# Autodesk Inventor assembly: Traction_Section_MIR2
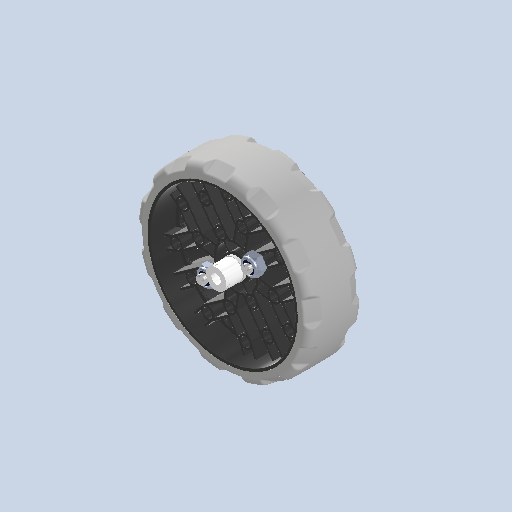
[picture p0: Inventor's stored thumbnail of the model, 512x512]
Saved by Autodesk Inventor 2025.2 (Build 292293000, 293)
## iProperties
Created: 2024-12-08
Part Number: Traction_Section_MIR2
Document SubType Name: Assembly
Designer: joshi
Author: Aditya Koduri
## Documents named in this file (11)
- C:\Users\joshi\Desktop\3388K CAD\Traction_Section_MIR2.iam
- C:\Users\joshi\Desktop\3388K CAD\VEX Main\Motion\Gears\HS Gear\HS 48T Gear, No Insert_MIR2.iam
- C:\Users\joshi\Desktop\3388K CAD\VEX Main\Structure\Hardware\Nut Thin Nylock_MIR2.ipt
- C:\Users\joshi\Desktop\3388K CAD\VEX Main\Motion\Insert Circle_MIR2.ipt
- C:\Users\joshi\Desktop\3388K CAD\VEX Main\Motion\Spacers\Washer Teflon\TWasher .375 OD x .03125.ipt
- C:\Users\joshi\Desktop\3388K CAD\VEX Main\Motion\Spacers\Washer Teflon.ipt
- C:\Users\joshi\Desktop\3388K CAD\VEX Main\Motion\Spacers\Spacer Nylon .313 OD\NSpacer .313 OD x .250.ipt
- C:\Users\joshi\Desktop\3388K CAD\VEX Main\Motion\Spacers\Spacer Nylon .313 OD.ipt
- C:\Users\joshi\Desktop\3388K CAD\VEX Main\Motion\Wheels\Traction Wheel\3.25 Traction AS, No Insert_MIR2.iam
- C:\Users\joshi\Desktop\3388K CAD\VEX Main\Structure\Hardware\Screw Steel - Hex\SScrew Hex Smooth 1.250.ipt
- C:\Users\joshi\Desktop\3388K CAD\VEX Main\Structure\Hardware\Screw Steel - Hex.ipt
## Components (13 placed, 7 different names)
1. HS 48T Gear, No Insert_MIR2:1 [sub-assembly] — Insert:7, Insert:14, Insert:15, Insert:16
2. Nut Thin Nylock_MIR2:1 — Insert:19
3. Nut Thin Nylock_MIR2:2 — Insert:18
4. Insert Circle_MIR2:1 — Insert:7, Insert:9
5. Insert Circle_MIR2:2 — Insert:12, Insert:17
6. TWasher .375 OD x .03125:1 — Insert:10
7. TWasher .375 OD x .03125:2 — Insert:10, Insert:9
8. NSpacer .313 OD x .250:1 — Insert:12, Insert:11
9. TWasher .375 OD x .03125:3 — Insert:11, Insert:13
10. TWasher .375 OD x .03125:4 — Insert:13
11. 3.25 Traction AS, No Insert_MIR2:1 [sub-assembly] — Insert:19, Insert:18, Insert:17, Insert:14
12. SScrew Hex Smooth 1.250:1 — Insert:15
13. SScrew Hex Smooth 1.250:2 — Insert:16
## Relationships (12: Insert 12)
- Insert:7: HS 48T Gear, No Insert_MIR2:1 ↔ Insert Circle_MIR2:1
- Insert:10: TWasher .375 OD x .03125:1 ↔ TWasher .375 OD x .03125:2
- Insert:9: Insert Circle_MIR2:1 ↔ TWasher .375 OD x .03125:2
- Insert:12: Insert Circle_MIR2:2 ↔ NSpacer .313 OD x .250:1
- Insert:11: NSpacer .313 OD x .250:1 ↔ TWasher .375 OD x .03125:3
- Insert:13: TWasher .375 OD x .03125:3 ↔ TWasher .375 OD x .03125:4
- Insert:19: Nut Thin Nylock_MIR2:1 ↔ 3.25 Traction AS, No Insert_MIR2:1
- Insert:18: Nut Thin Nylock_MIR2:2 ↔ 3.25 Traction AS, No Insert_MIR2:1
- Insert:17: Insert Circle_MIR2:2 ↔ 3.25 Traction AS, No Insert_MIR2:1
- Insert:14: HS 48T Gear, No Insert_MIR2:1 ↔ 3.25 Traction AS, No Insert_MIR2:1
- Insert:15: HS 48T Gear, No Insert_MIR2:1 ↔ SScrew Hex Smooth 1.250:1
- Insert:16: HS 48T Gear, No Insert_MIR2:1 ↔ SScrew Hex Smooth 1.250:2
